# Autodesk Inventor assembly: PKWS1
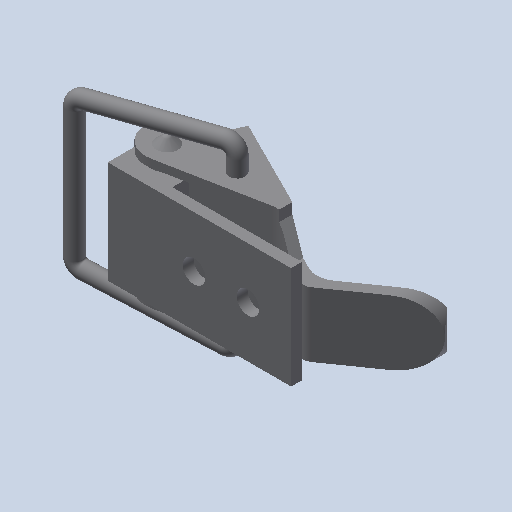
[picture p0: Inventor's stored thumbnail of the model, 512x512]
Saved by Autodesk Inventor 2024.2 (Build 282272000, 272)
## iProperties
Category: PARTsolutions
Company: MISUMI
Created: 2024-01-05
Part Number: PKWS1
Catalog Web Link: https://jp.misumi-ec.com/vona2/detail/110300523720/?ProductCode=PKWS1
Description: PKWS-Snap Locks
Vendor: MISUMI
Document SubType Name: Assembly
Designer: psAdmin
Manufacturer: MISUMI
Mass: 0.834159 g
Surface Area: 15.9556 cm^2
Volume: 0.834159 cm^3
Density: 1 g/cm^3
PSOL_IDENT_0: {$CADENAS_DATA/23d-libs/misumi/metric/44_handles_hinges/pkws_assmtab.prj},153 {VTYP=3D},{STYP=ASSTAB
PSOL_IDENT_1: },{NB=PKWS1},{LINA=PKWS1},{NN=PKWS},{DATE=04.06.2021 03:58:34},{GEOMDATE=17.02.2014},{VERSION=},{LIN
PSOL_IDENT_2: EID=10},{WBVAR=},{WBNUMERIC=}  {NB=PKWS1},{LINA=PKWS1},{KT=DUMMY},{PN=PKWS1},{MAT=304 Stainless Stee
PSOL_IDENT_3: l},{ST=Buffing},{NO=1},{TL=49 (5)},{MASS=6},{PPATH=pkws_templ.prj},{ANGLE=10.015}
NB: PKWS1
NN: PKWS
NT: Snap Locks
NBSYN: $PN.
LINA: PKWS1
CATALOG: Misumi
PN: PKWS1
MAT: 304 Stainless Steel
ST: Buffing
NO: 1
TL: 49 (5)
MASS: 6
SUPPLIER: MISUMI
ARTICLENO: PKWS1
BOMINFO: PKWS1
CREATOR: CADENAS GmbH
Title: PKWS1
Author: Cadenas PARTsolutions
Comments: Snap Locks
## Documents named in this file (4)
- C:\Users\masato\OneDrive - Chiba Institute of Technology\CIT Brains\RoboCup2024\Mechanic\SUSTAINA-OP2\NativeFiles\Boby\COTS\MisumiComponents\PKWS1.iam
- C:\Users\masato\OneDrive - Chiba Institute of Technology\CIT Brains\RoboCup2024\Mechanic\SUSTAINA-OP2\NativeFiles\Boby\COTS\MisumiComponents\PKWS1_b.ipt
- C:\Users\masato\OneDrive - Chiba Institute of Technology\CIT Brains\RoboCup2024\Mechanic\SUSTAINA-OP2\NativeFiles\Boby\COTS\MisumiComponents\PKWS1-HOOK.ipt
- C:\Users\masato\OneDrive - Chiba Institute of Technology\CIT Brains\RoboCup2024\Mechanic\SUSTAINA-OP2\NativeFiles\Boby\COTS\MisumiComponents\PKWS1-PIN.ipt
## Components (3 placed, 3 different names)
1. PKWS1_b:1 — A_XY@1 <-> A_XY@2, A_Z@1 <-> A_Z@2
2. PKWS1-HOOK:1 — A_XY@1 <-> A_XY@2, A_Z@1 <-> A_Z@2, B_XY@2 <-> B_XY@3, B_Z@2 <-> B_Z@3
3. PKWS1-PIN:1 — B_XY@2 <-> B_XY@3, B_Z@2 <-> B_Z@3
## Relationships (4: Flush 2, Mate 2)
- A_XY@1 <-> A_XY@2 [Flush]: PKWS1_b:1 ↔ PKWS1-HOOK:1
- A_Z@1 <-> A_Z@2 [Mate]: PKWS1_b:1 ↔ PKWS1-HOOK:1
- B_XY@2 <-> B_XY@3 [Flush]: PKWS1-HOOK:1 ↔ PKWS1-PIN:1
- B_Z@2 <-> B_Z@3 [Mate]: PKWS1-HOOK:1 ↔ PKWS1-PIN:1
